# Autodesk Inventor assembly: HbthumbU02ForChild_MIR1
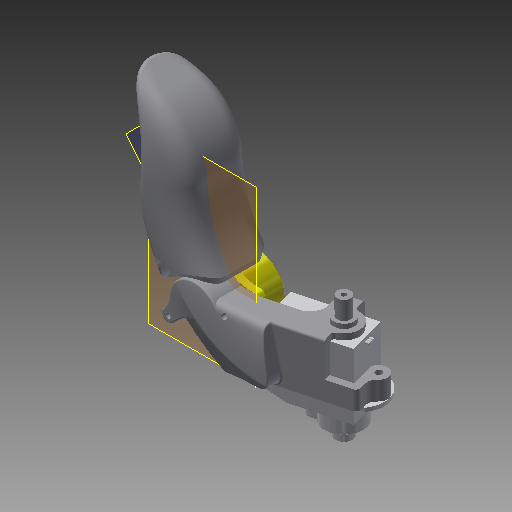
[picture p0: Inventor's stored thumbnail of the model, 512x512]
Saved by Autodesk Inventor 2017.3 (Build 213256000, 256)
## iProperties
Part Number: HbthumbU02ForChild_MIR1
Material: 一般
Document SubType Name: Assembly
Designer: sktom
Author: sktom
## Documents named in this file (8)
- D:\CloudStrage\OneDrive\CAD\MAJ\hackberry\HACKberry-hardware\3D_69%inlength\Inventor\HbHandForChild\HbthumbU02ForChild\HbthumbU02ForChild_MIR1.iam
- D:\CloudStrage\OneDrive\CAD\MAJ\hackberry\HACKberry-hardware\3D_69%inlength\Inventor\HbHandForChild\HbthumbU02ForChild\HbThumbMetacarpalPhalanx02ForChild_MIR1.ipt
- D:\CloudStrage\OneDrive\CAD\MAJ\hackberry\HACKberry-hardware\3D_69%inlength\Inventor\HbHandForChild\HbthumbU02ForChild\HbThumbLockButton01ForChild_MIR1.ipt
- D:\CloudStrage\OneDrive\CAD\MAJ\hackberry\HACKberry-hardware\3D_69%inlength\Inventor\HbHandForChild\HbthumbU02ForChild\HbThumbJointHolder01ForChild_MIR1.ipt
- D:\CloudStrage\OneDrive\CAD\MAJ\hackberry\HACKberry-hardware\3D_69%inlength\Inventor\HbHandForChild\HbthumbU02ForChild\HbThumbProximalPhalanx02ForChild_MIR1.ipt
- D:\CloudStrage\OneDrive\CAD\MAJ\hackberry\HACKberry-hardware\3D_69%inlength\Inventor\HbHandForChild\HbthumbU02ForChild\HbThumbProximalPhalanxBase02ForChild_MIR1.ipt
- D:\CloudStrage\OneDrive\CAD\MAJ\hackberry\HACKberry-hardware\3D_69%inlength\Inventor\HbHandForChild\HbthumbU02ForChild\HbThumbMetacarpalPhalanxCover02ForChild_MIR1.ipt
- D:\CloudStrage\OneDrive\CAD\MAJ\hackberry\HACKberry-hardware\3D_69%inlength\Inventor\HbHandForChild\HbthumbU02ForChild\HbServoHK282A\Servo_HK282A_MIR1.ipt
## Components (7 placed, 7 different names)
1. HbThumbMetacarpalPhalanx02ForChild_MIR1:1 — 挿入:3, 挿入:2, 挿入:1, 挿入:8, 挿入:7
2. HbThumbLockButton01ForChild_MIR1:1 — 挿入:3
3. HbThumbJointHolder01ForChild_MIR1:1 — 挿入:2, 挿入:1, 挿入:4, 挿入:6
4. HbThumbProximalPhalanx02ForChild_MIR1:1 — 挿入:5
5. HbThumbProximalPhalanxBase02ForChild_MIR1:1 — 挿入:5, 挿入:4
6. HbThumbMetacarpalPhalanxCover02ForChild_MIR1:1 — 挿入:6
7. Servo_HK282A_MIR1:1 — 挿入:8, 挿入:7
## Relationships (8: Insert 8)
- 挿入:3 [Insert] (2 mm): HbThumbMetacarpalPhalanx02ForChild_MIR1:1 ↔ HbThumbLockButton01ForChild_MIR1:1
- 挿入:2 [Insert]: HbThumbMetacarpalPhalanx02ForChild_MIR1:1 ↔ HbThumbJointHolder01ForChild_MIR1:1
- 挿入:1 [Insert]: HbThumbMetacarpalPhalanx02ForChild_MIR1:1 ↔ HbThumbJointHolder01ForChild_MIR1:1
- 挿入:5 [Insert] (0.2 mm): HbThumbProximalPhalanx02ForChild_MIR1:1 ↔ HbThumbProximalPhalanxBase02ForChild_MIR1:1
- 挿入:4 [Insert]: HbThumbJointHolder01ForChild_MIR1:1 ↔ HbThumbProximalPhalanxBase02ForChild_MIR1:1
- 挿入:6 [Insert]: HbThumbJointHolder01ForChild_MIR1:1 ↔ HbThumbMetacarpalPhalanxCover02ForChild_MIR1:1
- 挿入:8 [Insert]: HbThumbMetacarpalPhalanx02ForChild_MIR1:1 ↔ Servo_HK282A_MIR1:1
- 挿入:7 [Insert]: HbThumbMetacarpalPhalanx02ForChild_MIR1:1 ↔ Servo_HK282A_MIR1:1
